# Autodesk Inventor assembly: full
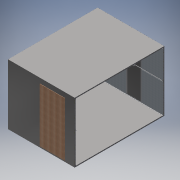
[picture p0: Inventor's stored thumbnail of the model, 180x180]
Saved by Autodesk Inventor 2019 (Build 230136000, 136)
## iProperties
Created: 2018-07-10
Part Number: full
Document SubType Name: Assembly
Designer: User
Author: User
## Documents named in this file (12)
- C:\Users\User\Documents\GitHub\darkRadio\3D Models\Room Model\full.iam
- C:\Users\User\Documents\GitHub\darkRadio\3D Models\Room Model\Room.ipt
- C:\Users\User\Documents\GitHub\darkRadio\3D Models\Room Model\left.iam
- C:\Users\User\Documents\GitHub\darkRadio\3D Models\Room Model\back.iam
- C:\Users\User\Documents\GitHub\darkRadio\3D Models\Room Model\right.iam
- C:\Users\User\Documents\GitHub\darkRadio\3D Models\Room Model\outlets.iam
- C:\Users\User\Documents\GitHub\darkRadio\3D Models\Room Model\gusset_frame.iam
- C:\Users\User\Documents\GitHub\darkRadio\3D Models\Room Model\door_rim.ipt
- C:\Users\User\Documents\GitHub\darkRadio\3D Models\Room Model\connection_plate.ipt
- C:\Users\User\Documents\GitHub\darkRadio\3D Models\Room Model\light.ipt
- C:\Users\User\Documents\GitHub\darkRadio\3D Models\Room Model\door.iam
- C:\Users\User\Documents\GitHub\darkRadio\3D Models\Room Model\params.xlsx
## Components (15 placed, 10 different names)
1. Room:1 — Planar:1, Planar:2, Planar:3, Planar:4, Planar:5, Planar:6, Planar:7, Planar:8, Planar:9, Planar:10, Flush:2, Mate:2, Mate:3, Mate:4, Mate:5, Rigid:2, Mate:6, Mate:7, Mate:8, Mate:9, Mate:11, Rigid:3
2. left:1 [sub-assembly] — Planar:1, Planar:2, Planar:3
3. back:1 [sub-assembly] — Planar:4, Planar:5, Planar:6
4. right:1 [sub-assembly] — Planar:7, Planar:8, Planar:9
5. outlets:1 [sub-assembly] — Planar:10, Flush:2, Mate:5
6. gusset_frame:1 [sub-assembly] — Mate:2, Mate:3, Mate:4, Mate:10
7. door_rim:1 — Rigid:2
8. connection_plate:1 — Mate:6, Mate:7, Mate:8
9. door:1 [sub-assembly] — Rigid:3
10. light:1 — Mate:9, Mate:10, Mate:11
11. light:2
12. light:3
13. light:4
14. light:5
15. light:6
## Component patterns: (6 elements, first: light:1)
## Relationships (23: PlanarJoint 10, Mate 10, WeldJoint 2, Flush 1)
- Planar:1 (25.4 mm): Room:1 ↔ left:1
- Planar:2 (25.4 mm): Room:1 ↔ left:1
- Planar:3: Room:1 ↔ left:1
- Planar:4 (31.75 mm): Room:1 ↔ back:1
- Planar:5 (25.4 mm): Room:1 ↔ back:1
- Planar:6: Room:1 ↔ back:1
- Planar:7 (38.1 mm): Room:1 ↔ right:1
- Planar:8 (25.4 mm): Room:1 ↔ right:1
- Planar:9: Room:1 ↔ right:1
- Planar:10: Room:1 ↔ outlets:1
- Flush:2 (-1320.8 mm): Room:1 ↔ outlets:1
- Mate:2: Room:1 ↔ gusset_frame:1
- Mate:3: Room:1 ↔ gusset_frame:1
- Mate:4: Room:1 ↔ gusset_frame:1
- Mate:5: Room:1 ↔ outlets:1
- Rigid:2 [WeldJoint]: Room:1 ↔ door_rim:1
- Mate:6: Room:1 ↔ connection_plate:1
- Mate:7 (257.175 mm): Room:1 ↔ connection_plate:1
- Mate:8 (190.5 mm): Room:1 ↔ connection_plate:1
- Mate:9 (20 mm): Room:1 ↔ light:1
- Mate:10 (1016 mm): gusset_frame:1 ↔ light:1
- Mate:11 (914.4 mm): Room:1 ↔ light:1
- Rigid:3 [WeldJoint]: Room:1 ↔ door:1
## Named parameters: wallThick = 44.45 mm, roomWidth = 3048 mm, roomDepth = 3657.6 mm, roomHeight = 2438.4 mm, doorWidth = 895.35 mm, doorHeight = 2108.2 mm, doorX = 774.7 mm, doorY = 88.9 mm, doorLip = 76.2 mm, doorThick = 57.15 mm, tubeD = 19.05 mm, tubeTurnR = 76.2 mm
